# Autodesk Inventor assembly: Camera_Mount
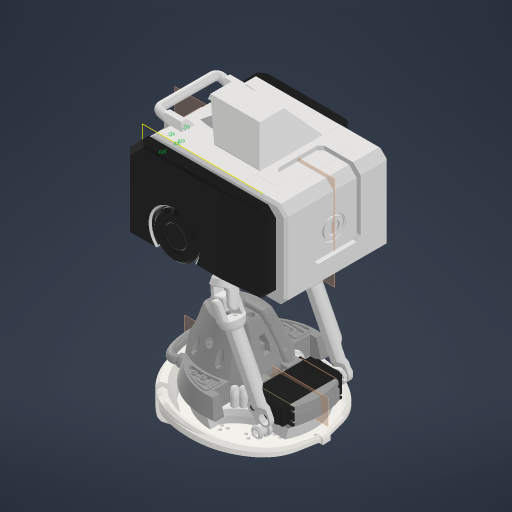
[picture p0: Inventor's stored thumbnail of the model, 512x512]
Saved by Autodesk Inventor 2024 (Build 280153000, 153)
## iProperties
Created: 2025-09-09
Part Number: Camera_Mount
Document SubType Name: Assembly
Designer: kevin
Author: kevin
## Documents named in this file (16)
- C:\Users\kevin\Desktop\Camera_Mount.iam
- C:\Users\kevin\Desktop\Camera_Baseplate.ipt
- C:\Users\kevin\Desktop\Camera_Gearplate.ipt
- C:\Users\kevin\Desktop\Neck_Cover.ipt
- C:\Users\kevin\Desktop\SeniorDesign\MG996R.ipt
- C:\Users\kevin\Desktop\SeniorDesign\Shaft_Long.ipt
- C:\Users\kevin\Desktop\Servo_Pulley.ipt
- C:\Users\kevin\Desktop\SeniorDesign\Universal_Joint.iam
- C:\Users\kevin\Desktop\SeniorDesign\Universal_Joint_Connector.ipt
- C:\Users\kevin\Desktop\SeniorDesign\Universal_Joint.ipt
- C:\Users\kevin\Desktop\SeniorDesign\Head_Baseplate.ipt
- C:\Users\kevin\Desktop\Camera_Mount\Design Accelerator\Spur Gears1.iam
- C:\Users\kevin\Desktop\Camera_Mount\Design Accelerator\Spur Gears2.iam
- C:\Users\kevin\Desktop\SeniorDesign\Gear_Cover.ipt
- C:\Users\kevin\Desktop\SeniorDesign\HEAD_PROTOTYPE_BOX.ipt
- C:\Users\kevin\Desktop\SeniorDesign\Head_V3\Head_V3_Assembly.iam
## Components (23 placed, 13 different names)
1. Camera_Baseplate:1 — Flush:2, Mate:1, Mate:4, Mate:5, Mate:6, Mate:7, Flush:4, Flush:5, Mate:15, Mate:16, Mate:17, Flush:15
2. Camera_Gearplate:1 — Mate:1, Flush:12, Mate:26, Mate:28, Mate:30, Mate:31
3. Neck_Cover:1 — Flush:2, Mate:18, Flush:8, Mate:19
4. MG996R:1 — Mate:4, Mate:5, Flush:5, Mate:32, Flush:13
5. MG996R:2 — Mate:6, Mate:7, Flush:4, Mate:10, Flush:6
6. Shaft_Long:1 — Mate:11, Mate:12, Mate:20, Flush:9, Mate:21
7. Servo_Pulley:1 — Mate:10, Flush:6, Mate:11, Mate:12
8. MG996R:3 — Mate:15, Mate:16, Mate:17, Flush:12, Mate:27, Mate:29
9. Universal_Joint:2 [sub-assembly] — Mate:18, Flush:8, Mate:19, Flush:10
10. Universal_Joint_Connector:1 — Mate:20, Flush:9, Mate:21, Mate:22, Mate:23
11. Universal_Joint_Connector:2 — Mate:24, Mate:25, Flush:11
12. Universal_Joint:3 — Mate:22, Mate:23, Mate:24, Mate:25
13. Head_Baseplate:1 — Flush:10, Flush:11, Mate:41, Mate:42
14. Spur Gears:1 [sub-assembly] — Mate:26, Mate:27
15. Spur Gears:2 [sub-assembly] — Mate:28, Mate:29, Mate:30, Mate:31
16. Shaft_Long:2 — Mate:33, Mate:34, Mate:39, Mate:40, Flush:14
17. Servo_Pulley:2 — Mate:32, Flush:13, Mate:33, Mate:34
18. Universal_Joint_Connector:3 — Mate:35, Mate:36, Mate:39, Mate:40, Flush:14
19. Universal_Joint_Connector:4 — Mate:37, Mate:38
20. Universal_Joint:4 — Mate:35, Mate:36, Mate:37, Mate:38
21. Gear_Cover:1 — Flush:15
22. HEAD_PROTOTYPE_BOX:1
23. Head_V3_Assembly:1 [sub-assembly] — Mate:41, Mate:42
## Relationships (48: Mate 36, Flush 12)
- Flush:2: Camera_Baseplate:1 ↔ Neck_Cover:1
- Mate:1: Camera_Baseplate:1 ↔ Camera_Gearplate:1
- Mate:4: Camera_Baseplate:1 ↔ MG996R:1
- Mate:5: Camera_Baseplate:1 ↔ MG996R:1
- Mate:6: Camera_Baseplate:1 ↔ MG996R:2
- Mate:7: Camera_Baseplate:1 ↔ MG996R:2
- Flush:4: Camera_Baseplate:1 ↔ MG996R:2
- Flush:5: Camera_Baseplate:1 ↔ MG996R:1
- Mate:10: MG996R:2 ↔ Servo_Pulley:1
- Flush:6: MG996R:2 ↔ Servo_Pulley:1
- Mate:11: Shaft_Long:1 ↔ Servo_Pulley:1
- Mate:12: Shaft_Long:1 ↔ Servo_Pulley:1
- Mate:15: Camera_Baseplate:1 ↔ MG996R:3
- Mate:16: Camera_Baseplate:1 ↔ MG996R:3
- Mate:17: Camera_Baseplate:1 ↔ MG996R:3
- Mate:18: Neck_Cover:1 ↔ Universal_Joint:2
- Flush:8: Neck_Cover:1 ↔ Universal_Joint:2
- Mate:19: Neck_Cover:1 ↔ Universal_Joint:2
- Mate:20: Shaft_Long:1 ↔ Universal_Joint_Connector:1
- Flush:9: Shaft_Long:1 ↔ Universal_Joint_Connector:1
- Mate:21: Shaft_Long:1 ↔ Universal_Joint_Connector:1
- Mate:22: Universal_Joint_Connector:1 ↔ Universal_Joint:3
- Mate:23 (0.3 mm): Universal_Joint_Connector:1 ↔ Universal_Joint:3
- Mate:24: Universal_Joint_Connector:2 ↔ Universal_Joint:3
- Mate:25 (0.3 mm): Universal_Joint_Connector:2 ↔ Universal_Joint:3
- Flush:10: Universal_Joint:2 ↔ Head_Baseplate:1
- Flush:11: Universal_Joint_Connector:2 ↔ Head_Baseplate:1
- Flush:12: Camera_Gearplate:1 ↔ MG996R:3
- Mate:26: Camera_Gearplate:1 ↔ Spur Gears:1
- Mate:27: MG996R:3 ↔ Spur Gears:1
- Mate:28: Camera_Gearplate:1 ↔ Spur Gears:2
- Mate:29: MG996R:3 ↔ Spur Gears:2
- Mate:30: Camera_Gearplate:1 ↔ Spur Gears:2
- Mate:31: Camera_Gearplate:1 ↔ Spur Gears:2
- Mate:32: MG996R:1 ↔ Servo_Pulley:2
- Flush:13: MG996R:1 ↔ Servo_Pulley:2
- Mate:33: Shaft_Long:2 ↔ Servo_Pulley:2
- Mate:34: Shaft_Long:2 ↔ Servo_Pulley:2
- Mate:35: Universal_Joint_Connector:3 ↔ Universal_Joint:4
- Mate:36 (0.3 mm): Universal_Joint_Connector:3 ↔ Universal_Joint:4
- Mate:37: Universal_Joint_Connector:4 ↔ Universal_Joint:4
- Mate:38 (0.3 mm): Universal_Joint_Connector:4 ↔ Universal_Joint:4
- Mate:39: Shaft_Long:2 ↔ Universal_Joint_Connector:3
- Mate:40: Shaft_Long:2 ↔ Universal_Joint_Connector:3
- Flush:14: Shaft_Long:2 ↔ Universal_Joint_Connector:3
- Flush:15: Camera_Baseplate:1 ↔ Gear_Cover:1
- Mate:41: Head_Baseplate:1 ↔ Head_V3_Assembly:1
- Mate:42: Head_Baseplate:1 ↔ Head_V3_Assembly:1
